# Autodesk Inventor assembly: Assembly1
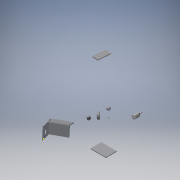
[picture p0: Inventor's stored thumbnail of the model, 180x180]
Saved by Autodesk Inventor 2019 (Build 230136000, 136)
## iProperties
Created: 2020-02-19
Part Number: Assembly1
Document SubType Name: Assembly
Designer: unusualgamer
Author: unusualgamer
## Documents named in this file (10)
- D:\New Folder\Assembly1.iam
- D:\New Folder\cutter grp 17-1.ipt
- D:\New Folder\cutter grp 17-2.ipt
- D:\New Folder\Motor DC.ipt
- D:\New Folder\roller1 grp17.ipt
- D:\New Folder\roller2 grp17.ipt
- D:\New Folder\roller3 grp17.ipt
- C:\Users\unusualgamer\OneDrive\Documents\side.ipt
- C:\Users\unusualgamer\OneDrive\Documents\bottom.ipt
- C:\Users\unusualgamer\OneDrive\Documents\front.ipt
## Components (11 placed, 9 different names)
1. cutter grp 17-1:1
2. cutter grp 17-2:1
3. Motor DC:1
4. roller1 grp17:1
5. roller2 grp17:1
6. roller3 grp17:1
7. side:1
8. side:2
9. bottom:1 — Mate:1, Mate:2
10. front:1 — Mate:2
11. bottom:2 — Mate:1
## Relationships (2: Mate 2)
- Mate:1: bottom:1 ↔ bottom:2
- Mate:2: bottom:1 ↔ front:1
